# Autodesk Inventor assembly: Auto_robot_gate_mechanism_V1_11.10.25
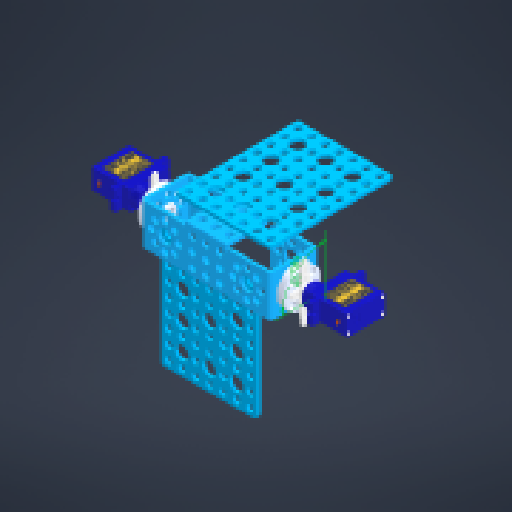
[picture p0: Inventor's stored thumbnail of the model, 512x512]
Saved by Autodesk Inventor 2026.1 (Build 301233020, 233B)
## iProperties
Created: 2025-10-11
Part Number: Auto_robot_gate_mechanism_V1_11.10.25
Document SubType Name: Assembly
Designer: Asus
Author: Asus
## Documents named in this file (7)
- D:\KMITL\Computer_Programming\ComPro_Project\Robot_design_CAD_files\Auto_robot_gate_mechanism_V1_11.10.25.iam
- D:\KMITL\Computer_Programming\ComPro_Project\Material_Parts_CAD_files\Metal_parts\U-Shape_Bracket.ipt
- D:\KMITL\Computer_Programming\ComPro_Project\Material_Parts_CAD_files\Metal_parts\Bracket 3x3.ipt
- D:\KMITL\Computer_Programming\ComPro_Project\Material_Parts_CAD_files\Metal_parts\Plate 7x9.ipt
- D:\KMITL\Computer_Programming\ComPro_Project\Material_Parts_CAD_files\MakeX_parts\Shaft Connector.ipt
- D:\KMITL\Computer_Programming\ComPro_Project\Material_Parts_CAD_files\Electronic_parts\SG90 - Micro Servo 9g.ipt
- D:\KMITL\Computer_Programming\ComPro_Project\Material_Parts_CAD_files\Electronic_parts\Micro Servo 9g connector.ipt
## Components (11 placed, 6 different names)
1. U-Shape_Bracket:1 — Rigid:3, Rigid:5
2. Bracket 3x3:1 — Rigid:1, Rigid:2
3. Plate 7x9:1 — Rigid:1
4. Plate 7x9:2 — Rigid:2, Rigid:3, Rigid:4
5. U-Shape_Bracket:2 — Rigid:4, Rigid:6
6. Shaft Connector:1 — Rigid:5, Rigid:7
7. Shaft Connector:2 — Rigid:6, Rigid:8
8. SG90 - Micro Servo 9g:1 — Rotational:1, Mate:2
9. Micro Servo 9g connector:1 — Rigid:7, Rotational:1
10. SG90 - Micro Servo 9g:2 — Rotational:2, Mate:3, Mate:4
11. Micro Servo 9g connector:2 — Rigid:8, Rotational:2
## Relationships (13: WeldJoint 8, Mate 3, RevoluteJoint 2)
- Rigid:1 [WeldJoint]: Bracket 3x3:1 ↔ Plate 7x9:1
- Rigid:2 [WeldJoint]: Bracket 3x3:1 ↔ Plate 7x9:2
- Rigid:3 [WeldJoint]: U-Shape_Bracket:1 ↔ Plate 7x9:2
- Rigid:4 [WeldJoint]: Plate 7x9:2 ↔ U-Shape_Bracket:2
- Rigid:5 [WeldJoint]: U-Shape_Bracket:1 ↔ Shaft Connector:1
- Rigid:6 [WeldJoint]: U-Shape_Bracket:2 ↔ Shaft Connector:2
- Rigid:7 [WeldJoint]: Shaft Connector:1 ↔ Micro Servo 9g connector:1
- Rigid:8 [WeldJoint]: Shaft Connector:2 ↔ Micro Servo 9g connector:2
- Rotational:1 [RevoluteJoint]: SG90 - Micro Servo 9g:1 ↔ Micro Servo 9g connector:1
- Rotational:2 [RevoluteJoint]: SG90 - Micro Servo 9g:2 ↔ Micro Servo 9g connector:2
- Mate:2: SG90 - Micro Servo 9g:1
- Mate:3: SG90 - Micro Servo 9g:2
- Mate:4: SG90 - Micro Servo 9g:2
